# Autodesk Inventor assembly: sensory_platform
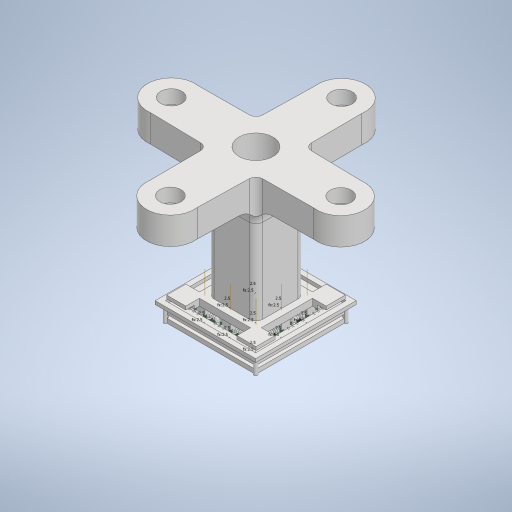
[picture p0: Inventor's stored thumbnail of the model, 512x512]
Saved by Autodesk Inventor 2023.1 (Build 271208000, 208)
## iProperties
Created: 2022-08-08
Part Number: sensory_platform
Document SubType Name: Assembly
Designer: fraaw
Author: fraaw
## Documents named in this file (5)
- C:\Users\fraaw\OneDrive\Desktop\sensory_platform.iam
- C:\Users\fraaw\OneDrive\Desktop\franka_mount.ipt
- C:\Users\fraaw\OneDrive\Desktop\sensor_soldering_mold.ipt
- C:\Users\fraaw\OneDrive\Desktop\sensor_holder.ipt
- C:\Users\fraaw\OneDrive\Desktop\sensor_unit.ipt
## Components (12 placed, 4 different names)
1. franka_mount:1 — Rigid:1
2. sensor_soldering_mold:1
3. sensor_holder:1 — Rigid:1, Rigid:2
4. sensor_unit:1 — Rigid:2
5. sensor_unit:2
6. sensor_unit:3
7. sensor_unit:4
8. sensor_unit:5
9. sensor_unit:6
10. sensor_unit:7
11. sensor_unit:8
12. sensor_unit:9
## Component patterns: (9 elements, first: sensor_unit:1)
## Relationships (2: WeldJoint 2)
- Rigid:1 [WeldJoint] (-5 mm): franka_mount:1 ↔ sensor_holder:1
- Rigid:2 [WeldJoint]: sensor_holder:1 ↔ sensor_unit:1
